# Autodesk Inventor assembly: SAR330 + regular couplers NG
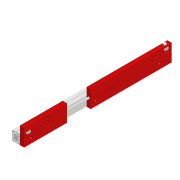
[picture p0: Inventor's stored thumbnail of the model, 180x180]
Saved by Autodesk Inventor 2020 (Build 240168000, 168)
## iProperties
Created: 2019-11-17
Part Number: SAR330 + regular couplers NG
Document SubType Name: Assembly
Designer: ball
Author: ball
## Documents named in this file (5)
- C:\FTC\FTC8863CAD\2019 Robot\Delivery\SAR330 + regular couplers.iam
- C:\FTC\FTC8863CAD\Misumi\SAR330\SAR330.iam
- C:\FTC\FTC8863CAD\2019 Robot\Delivery\Coupler bottom regular + pulleys.iam
- C:\FTC\FTC8863CAD\Actobotics\634 parts\634266.ipt
- C:\FTC\FTC8863CAD\2019 Robot\Delivery\Coupler top regular + pulleys.iam
## Components (4 placed, 4 different names)
1. SAR330:1 [sub-assembly] — Mate:1, Mate:2, Angle:1, Mate:5, Mate:6, Mate:7
2. Coupler bottom regular + pulleys:1 [sub-assembly] — Mate:1, Mate:2, Angle:1, Mate:3, Mate:4
3. 634266:1 — Mate:3, Mate:4
4. Coupler top regular + pulleys:1 [sub-assembly] — Mate:5, Mate:6, Mate:7
## Relationships (8: Mate 7, Angle 1)
- Mate:1: SAR330:1 ↔ Coupler bottom regular + pulleys:1
- Mate:2: SAR330:1 ↔ Coupler bottom regular + pulleys:1
- Angle:1 (0 deg): SAR330:1 ↔ Coupler bottom regular + pulleys:1
- Mate:3: Coupler bottom regular + pulleys:1 ↔ 634266:1
- Mate:4: Coupler bottom regular + pulleys:1 ↔ 634266:1
- Mate:5: SAR330:1 ↔ Coupler top regular + pulleys:1
- Mate:6: SAR330:1 ↔ Coupler top regular + pulleys:1
- Mate:7: SAR330:1 ↔ Coupler top regular + pulleys:1
